# Autodesk Inventor assembly: Ensamblaje
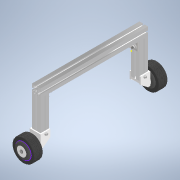
[picture p0: Inventor's stored thumbnail of the model, 180x180]
Saved by Autodesk Inventor 2021 (Build 250183000, 183)
## iProperties
Created: 2021-01-22
Part Number: Ensamblaje
Document SubType Name: Assembly
Designer: juanm
Author: juanm
## Documents named in this file (13)
- C:\Users\juanm\OneDrive\Documentos\Inventor\Rembot - Locomoción\Ensamblaje.iam
- C:\Users\juanm\OneDrive\Documentos\Inventor\Rembot - Locomoción\Horizontal.ipt
- C:\Users\juanm\OneDrive\Documentos\Inventor\Rembot - Locomoción\Vertical.ipt
- C:\Users\juanm\OneDrive\Documentos\Inventor\Rembot - Locomoción\Sujetador.ipt
- C:\Users\juanm\OneDrive\Documentos\Inventor\Rembot - Locomoción\TornilloM8.ipt
- C:\Users\juanm\OneDrive\Documentos\Inventor\Rembot - Locomoción\Tuerca para tornilloM8.ipt
- C:\Users\juanm\OneDrive\Documentos\Inventor\Rembot - Locomoción\TornilloM6.ipt
- C:\Users\juanm\OneDrive\Documentos\Inventor\Rembot - Locomoción\UnionLlantaOmega.ipt
- C:\Users\juanm\OneDrive\Documentos\Inventor\Rembot - Locomoción\Tuerca para tornilloM6.ipt
- C:\Users\juanm\OneDrive\Documentos\Inventor\Rembot - Locomoción\Socket.ipt
- C:\Users\juanm\OneDrive\Documentos\Inventor\Rembot - Locomoción\Llanta.ipt
- C:\Users\juanm\OneDrive\Documentos\Inventor\Rembot - Locomoción\Rondana.ipt
- C:\Users\juanm\OneDrive\Documentos\Inventor\Rembot - Locomoción\TuercaLlanta.ipt
## Components (31 placed, 12 different names)
1. Horizontal:1 — Coincidencia:1, Nivelación:1, Nivelación:2, Coincidencia:3, Nivelación:3, Coincidencia:7, Coincidencia:8, Coincidencia:9, Coincidencia:10, Coincidencia:11, Coincidencia:12, Coincidencia:13, Coincidencia:14, Coincidencia:15, Nivelación:4, Nivelación:5, Coincidencia:16, Coincidencia:17, Coincidencia:18, Coincidencia:22
2. Vertical:1 — Coincidencia:1, Nivelación:1, Nivelación:2, Coincidencia:2, Coincidencia:4, Coincidencia:5, Coincidencia:6, Coincidencia:32, Coincidencia:33, Coincidencia:34, Coincidencia:35, Coincidencia:36, Coincidencia:37, Nivelación:8, Coincidencia:38, Coincidencia:39, De rotación:10
3. Sujetador:1 — Coincidencia:2, Coincidencia:3, Nivelación:3
4. TornilloM8:1 — Coincidencia:4, Coincidencia:5, Coincidencia:6, De rotación:2
5. TornilloM8:2 — Coincidencia:7, Coincidencia:8, Coincidencia:9, De rotación:1
6. Tuerca para tornilloM8:1 — De rotación:2
7. Tuerca para tornilloM8:2 — De rotación:1
8. Vertical:2 — Coincidencia:15, Nivelación:4, Nivelación:5, Coincidencia:19, Coincidencia:20, Coincidencia:21, Nivelación:6, Coincidencia:23, Coincidencia:24, Coincidencia:25, Coincidencia:26, Coincidencia:27, Coincidencia:28, Coincidencia:29, Nivelación:7, Coincidencia:30, Coincidencia:31, De rotación:9
9. TornilloM8:3 — Coincidencia:19, Coincidencia:20, Coincidencia:21, De rotación:4
10. TornilloM8:4 — Coincidencia:16, Coincidencia:17, Coincidencia:18, De rotación:3
11. Sujetador:2 — Nivelación:6, Coincidencia:22, Coincidencia:23
12. Tuerca para tornilloM8:3 — De rotación:3
13. Tuerca para tornilloM8:4 — De rotación:4
14. TornilloM6:1 — Coincidencia:24, Coincidencia:25, Coincidencia:26, De rotación:5
15. TornilloM6:2 — Coincidencia:27, Coincidencia:28, Coincidencia:29, De rotación:6
16. UnionLlantaOmega:1 — Nivelación:7, Coincidencia:30, Coincidencia:31, Insertar:1
17. Tuerca para tornilloM6:1 — De rotación:6
18. Tuerca para tornilloM6:2 — De rotación:5
19. TornilloM6:3 — Coincidencia:35, Coincidencia:36, Coincidencia:37, De rotación:7
20. TornilloM6:4 — Coincidencia:32, Coincidencia:33, Coincidencia:34, De rotación:8
21. UnionLlantaOmega:2 — Nivelación:8, Coincidencia:38, Coincidencia:39, Insertar:2
22. Tuerca para tornilloM6:3 — De rotación:8
23. Tuerca para tornilloM6:4 — De rotación:7
24. Socket:1 — De rotación:10
25. Socket:2 — De rotación:9
26. Llanta:1 — Insertar:1, De rotación:11, De rotación:13
27. Llanta:2 — Insertar:2, De rotación:12, De rotación:14
28. Rondana:1 — De rotación:12
29. Rondana:2 — De rotación:11
30. TuercaLlanta:1 — De rotación:13
31. TuercaLlanta:2 — De rotación:14
## Relationships (63: Mate 39, RevoluteJoint 14, Flush 8, Insert 2)
- Coincidencia:1 [Mate]: Horizontal:1 ↔ Vertical:1
- Nivelación:1 [Flush]: Horizontal:1 ↔ Vertical:1
- Nivelación:2 [Flush]: Horizontal:1 ↔ Vertical:1
- Coincidencia:2 [Mate]: Vertical:1 ↔ Sujetador:1
- Coincidencia:3 [Mate]: Horizontal:1 ↔ Sujetador:1
- Nivelación:3 [Flush] (5 mm): Horizontal:1 ↔ Sujetador:1
- Coincidencia:4 [Mate] (-135.5 mm): Vertical:1 ↔ TornilloM8:1
- Coincidencia:5 [Mate]: Vertical:1 ↔ TornilloM8:1
- Coincidencia:6 [Mate] (2.3 mm): Vertical:1 ↔ TornilloM8:1
- Coincidencia:7 [Mate] (-434.5 mm): Horizontal:1 ↔ TornilloM8:2
- Coincidencia:8 [Mate]: Horizontal:1 ↔ TornilloM8:2
- Coincidencia:9 [Mate] (2.2 mm): Horizontal:1 ↔ TornilloM8:2
- De rotación:1 [RevoluteJoint] (-6.6 mm): TornilloM8:2 ↔ Tuerca para tornilloM8:2
- De rotación:2 [RevoluteJoint] (6.6 mm): TornilloM8:1 ↔ Tuerca para tornilloM8:1
- Coincidencia:10 [Mate]: Horizontal:1
- Coincidencia:11 [Mate]: Horizontal:1
- Coincidencia:12 [Mate]: Horizontal:1
- Coincidencia:13 [Mate]: Horizontal:1
- Coincidencia:14 [Mate]: Horizontal:1
- Coincidencia:15 [Mate]: Horizontal:1 ↔ Vertical:2
- Nivelación:4 [Flush]: Horizontal:1 ↔ Vertical:2
- Nivelación:5 [Flush]: Horizontal:1 ↔ Vertical:2
- Coincidencia:16 [Mate] (-72.5 mm): Horizontal:1 ↔ TornilloM8:4
- Coincidencia:17 [Mate]: Horizontal:1 ↔ TornilloM8:4
- Coincidencia:18 [Mate] (2.2 mm): Horizontal:1 ↔ TornilloM8:4
- Coincidencia:19 [Mate] (-135 mm): Vertical:2 ↔ TornilloM8:3
- Coincidencia:20 [Mate]: Vertical:2 ↔ TornilloM8:3
- Coincidencia:21 [Mate] (2.2 mm): Vertical:2 ↔ TornilloM8:3
- Nivelación:6 [Flush] (5 mm): Vertical:2 ↔ Sujetador:2
- Coincidencia:22 [Mate]: Horizontal:1 ↔ Sujetador:2
- Coincidencia:23 [Mate]: Vertical:2 ↔ Sujetador:2
- De rotación:3 [RevoluteJoint] (6.6 mm): TornilloM8:4 ↔ Tuerca para tornilloM8:3
- De rotación:4 [RevoluteJoint] (-6.6 mm): TornilloM8:3 ↔ Tuerca para tornilloM8:4
- Coincidencia:24 [Mate] (-13.1 mm): Vertical:2 ↔ TornilloM6:1
- Coincidencia:25 [Mate]: Vertical:2 ↔ TornilloM6:1
- Coincidencia:26 [Mate] (3.3 mm): Vertical:2 ↔ TornilloM6:1
- Coincidencia:27 [Mate] (-13.1 mm): Vertical:2 ↔ TornilloM6:2
- Coincidencia:28 [Mate]: Vertical:2 ↔ TornilloM6:2
- Coincidencia:29 [Mate] (3.3 mm): Vertical:2 ↔ TornilloM6:2
- Nivelación:7 [Flush] (-5 mm): Vertical:2 ↔ UnionLlantaOmega:1
- Coincidencia:30 [Mate]: Vertical:2 ↔ UnionLlantaOmega:1
- Coincidencia:31 [Mate]: Vertical:2 ↔ UnionLlantaOmega:1
- De rotación:5 [RevoluteJoint] (-1 mm): TornilloM6:1 ↔ Tuerca para tornilloM6:2
- De rotación:6 [RevoluteJoint] (1 mm): TornilloM6:2 ↔ Tuerca para tornilloM6:1
- Coincidencia:32 [Mate] (-13.1 mm): Vertical:1 ↔ TornilloM6:4
- Coincidencia:33 [Mate]: Vertical:1 ↔ TornilloM6:4
- Coincidencia:34 [Mate] (3.3 mm): Vertical:1 ↔ TornilloM6:4
- Coincidencia:35 [Mate] (-13.1 mm): Vertical:1 ↔ TornilloM6:3
- Coincidencia:36 [Mate]: Vertical:1 ↔ TornilloM6:3
- Coincidencia:37 [Mate] (3.3 mm): Vertical:1 ↔ TornilloM6:3
- Nivelación:8 [Flush] (-5 mm): Vertical:1 ↔ UnionLlantaOmega:2
- Coincidencia:38 [Mate]: Vertical:1 ↔ UnionLlantaOmega:2
- Coincidencia:39 [Mate]: Vertical:1 ↔ UnionLlantaOmega:2
- De rotación:7 [RevoluteJoint] (-1 mm): TornilloM6:3 ↔ Tuerca para tornilloM6:4
- De rotación:8 [RevoluteJoint] (1 mm): TornilloM6:4 ↔ Tuerca para tornilloM6:3
- De rotación:9 [RevoluteJoint] (-6 mm): Vertical:2 ↔ Socket:2
- De rotación:10 [RevoluteJoint] (6 mm): Vertical:1 ↔ Socket:1
- Insertar:1 (-20 mm): UnionLlantaOmega:1 ↔ Llanta:1
- Insertar:2 (-20 mm): UnionLlantaOmega:2 ↔ Llanta:2
- De rotación:11 [RevoluteJoint] (-7.5 mm): Llanta:1 ↔ Rondana:2
- De rotación:12 [RevoluteJoint] (-10 mm): Llanta:2 ↔ Rondana:1
- De rotación:13 [RevoluteJoint] (-2.5 mm): Llanta:1 ↔ TuercaLlanta:1
- De rotación:14 [RevoluteJoint] (-7.6 mm): Llanta:2 ↔ TuercaLlanta:2
